# Autodesk Inventor assembly: Chamber_assembly_vers_4
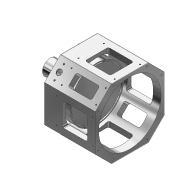
[picture p0: Inventor's stored thumbnail of the model, 180x180]
Saved by Autodesk Inventor 2013 (Build 170138000, 138)
## iProperties
Created: 2012-06-12
Part Number: Chamber_assembly_vers_4
Document SubType Name: Assembly
Designer: Breckenridge2 User
Author: Breckenridge2 User
## Documents named in this file (3)
- D:\Work_Suranga\3d_drawing_of_the_chamber\Educational_version\Chamber_assembly_vers_4.iam
- D:\Work_Suranga\3d_drawing_of_the_chamber\Chamber_drawings\Chamber_wall_NEW_v_6.ipt
- D:\Work_Suranga\3d_drawing_of_the_chamber\Educational_version\Electrode_assembly_v6.iam
## Components (2 placed, 2 different names)
1. Chamber_wall_NEW_v_6:1 — Insert:1, Insert:2, Insert:3
2. Electrode_assembly_v6:1 [sub-assembly] — Insert:1, Insert:2, Insert:3
## Relationships (3: Insert 3)
- Insert:1: Chamber_wall_NEW_v_6:1 ↔ Electrode_assembly_v6:1
- Insert:2: Chamber_wall_NEW_v_6:1 ↔ Electrode_assembly_v6:1
- Insert:3: Chamber_wall_NEW_v_6:1 ↔ Electrode_assembly_v6:1
